# Autodesk Inventor assembly: Wheel Assembly, Left
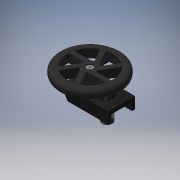
[picture p0: Inventor's stored thumbnail of the model, 180x180]
Saved by Autodesk Inventor 2017 (Build 210142000, 142)
## iProperties
Created: 2018-10-18
Part Number: Wheel Assembly, Left
Document SubType Name: Assembly
Designer: Dell
Author: Dell
## Documents named in this file (9)
- C:\Users\Dell\Documents\GitHub\tr2\Wheel Assembly\Wheel Assembly, Left.iam
- C:\Users\Dell\Documents\GitHub\tr2\Wheel Assembly\Scooter Wheel.ipt
- C:\Users\Dell\Documents\GitHub\tr2\Wheel Assembly\WA01.ipt
- C:\Users\Dell\Documents\GitHub\tr2\Wheel Assembly\Wheel Assembly\Design Accelerator\Spur Gears1.iam
- C:\Users\Dell\Documents\GitHub\tr2\Base\37d-gearmotor-50-70-encoder.ipt
- C:\Users\Dell\Documents\GitHub\tr2\Wheel Assembly\22x8x8mm Bearing.ipt
- C:\Users\Dell\Documents\GitHub\tr2\Wheel Assembly\6mm Mounting Hub, thin.ipt
- C:\Users\Dell\Documents\GitHub\tr2\Wheel Assembly\WA03.ipt
- C:\Users\Dell\Documents\GitHub\tr2\Wheel Assembly\WA04.ipt
## Components (13 placed, 8 different names)
1. Scooter Wheel:1 — Mate:25, Mate:26, Mate:27, Mate:28, Mate:47, Rotation:1
2. WA01:1 — Mate:9, Mate:10, Mate:11, Mate:36, Mate:39, Mate:40, Mate:42, Mate:43, Mate:44, Mate:46, Mate:62, Mate:66, Mate:67, Mate:68, Mate:69, Mate:70
3. Spur Gears:1 [sub-assembly] — Mate:21, Mate:22, Mate:44, Mate:45, Mate:46, Mate:47, Rotation:1, Mate:48, Mate:49, Mate:50
4. 37d-gearmotor-50-70-encoder:1 — Mate:9, Mate:10, Mate:11, Mate:20, Mate:45
5. 22x8x8mm Bearing:1 — Mate:37, Mate:48
6. 22x8x8mm Bearing:2 — Mate:36, Mate:37, Mate:49
7. 6mm Mounting Hub, thin:1 — Mate:20, Mate:21, Mate:22
8. 22x8x8mm Bearing:4 — Mate:25, Mate:26
9. 22x8x8mm Bearing:5 — Mate:27, Mate:28, Mate:50
10. 22x8x8mm Bearing:6 — Mate:39, Mate:40
11. 22x8x8mm Bearing:7 — Mate:42, Mate:43
12. WA04:1 — Mate:63, Mate:71
13. WA03:1 — Mate:62, Mate:63, Mate:69, Mate:70, Mate:71
## Relationships (32: Mate 31, RelateRotation 1)
- Mate:9: WA01:1 ↔ 37d-gearmotor-50-70-encoder:1
- Mate:10: WA01:1 ↔ 37d-gearmotor-50-70-encoder:1
- Mate:11: WA01:1 ↔ 37d-gearmotor-50-70-encoder:1
- Mate:20: 37d-gearmotor-50-70-encoder:1 ↔ 6mm Mounting Hub, thin:1
- Mate:21: Spur Gears:1 ↔ 6mm Mounting Hub, thin:1
- Mate:22: Spur Gears:1 ↔ 6mm Mounting Hub, thin:1
- Mate:25: Scooter Wheel:1 ↔ 22x8x8mm Bearing:4
- Mate:26: Scooter Wheel:1 ↔ 22x8x8mm Bearing:4
- Mate:27: Scooter Wheel:1 ↔ 22x8x8mm Bearing:5
- Mate:28: Scooter Wheel:1 ↔ 22x8x8mm Bearing:5
- Mate:36: WA01:1 ↔ 22x8x8mm Bearing:2
- Mate:37: 22x8x8mm Bearing:1 ↔ 22x8x8mm Bearing:2
- Mate:39: WA01:1 ↔ 22x8x8mm Bearing:6
- Mate:40: WA01:1 ↔ 22x8x8mm Bearing:6
- Mate:42: WA01:1 ↔ 22x8x8mm Bearing:7
- Mate:43: WA01:1 ↔ 22x8x8mm Bearing:7
- Mate:44: WA01:1 ↔ Spur Gears:1
- Mate:45: Spur Gears:1 ↔ 37d-gearmotor-50-70-encoder:1
- Mate:46: WA01:1 ↔ Spur Gears:1
- Mate:47: Scooter Wheel:1 ↔ Spur Gears:1
- Rotation:1 [RelateRotation] (1 ul): Scooter Wheel:1 ↔ Spur Gears:1
- Mate:48: Spur Gears:1 ↔ 22x8x8mm Bearing:1
- Mate:49: Spur Gears:1 ↔ 22x8x8mm Bearing:2
- Mate:50: Spur Gears:1 ↔ 22x8x8mm Bearing:5
- Mate:62: WA01:1 ↔ WA03:1
- Mate:63: WA04:1 ↔ WA03:1
- Mate:66: WA01:1
- Mate:67: WA01:1
- Mate:68: WA01:1
- Mate:69: WA01:1 ↔ WA03:1
- Mate:70: WA01:1 ↔ WA03:1
- Mate:71 (0.5 mm): WA04:1 ↔ WA03:1
